# Autodesk Inventor assembly: Pulley
Saved by Autodesk Inventor 2016 (Build 200138000, 138)
## iProperties
Created: 2017-01-08
Part Number: Pulley
Document SubType Name: Assembly
Designer: Dhruv
Author: Dhruv
## Documents named in this file (4)
- C:\Users\Dhruv\Desktop\MISC\FRC 2017\Pulley.iam
- C:\Users\Dhruv\Desktop\MISC\FRC 2017\supporting_parts\am-2234_42toothHTDpulleyHalfRev2.ipt
- C:\Users\Dhruv\Desktop\MISC\FRC 2017\supporting_parts\am-2568 500EX Hex Hub.ipt
- C:\Users\Dhruv\Desktop\MISC\FRC 2017\HubBoltWithLockNut.iam
## Components (9 placed, 3 different names)
1. am-2234_42toothHTDpulleyHalfRev2:1
2. am-2234_42toothHTDpulleyHalfRev2:2
3. am-2568 500EX Hex Hub:1
4. HubBoltWithLockNut:1 [sub-assembly]
5. HubBoltWithLockNut:2 [sub-assembly]
6. HubBoltWithLockNut:3 [sub-assembly]
7. HubBoltWithLockNut:4 [sub-assembly]
8. HubBoltWithLockNut:5 [sub-assembly]
9. HubBoltWithLockNut:6 [sub-assembly]
## Relationships (19: Mate 19)
- [Mate]: am-2234_42toothHTDpulleyHalfRev2:1 ↔ am-2234_42toothHTDpulleyHalfRev2:2
- [Mate]: am-2234_42toothHTDpulleyHalfRev2:1 ↔ am-2234_42toothHTDpulleyHalfRev2:2
- [Mate]: am-2234_42toothHTDpulleyHalfRev2:1 ↔ am-2234_42toothHTDpulleyHalfRev2:2
- [Mate]: am-2234_42toothHTDpulleyHalfRev2:1 ↔ am-2234_42toothHTDpulleyHalfRev2:2
- [Mate]: am-2234_42toothHTDpulleyHalfRev2:2 ↔ am-2568 500EX Hex Hub:1
- [Mate]: am-2234_42toothHTDpulleyHalfRev2:2 ↔ am-2568 500EX Hex Hub:1
- [Mate]: am-2234_42toothHTDpulleyHalfRev2:2 ↔ am-2568 500EX Hex Hub:1
- [Mate]: am-2568 500EX Hex Hub:1 ↔ HubBoltWithLockNut:1
- [Mate]: am-2568 500EX Hex Hub:1 ↔ HubBoltWithLockNut:1
- [Mate]: am-2568 500EX Hex Hub:1 ↔ HubBoltWithLockNut:2
- [Mate]: am-2568 500EX Hex Hub:1 ↔ HubBoltWithLockNut:2
- [Mate]: am-2568 500EX Hex Hub:1 ↔ HubBoltWithLockNut:3
- [Mate]: am-2568 500EX Hex Hub:1 ↔ HubBoltWithLockNut:3
- [Mate]: am-2568 500EX Hex Hub:1 ↔ HubBoltWithLockNut:6
- [Mate]: am-2568 500EX Hex Hub:1 ↔ HubBoltWithLockNut:6
- [Mate]: am-2568 500EX Hex Hub:1 ↔ HubBoltWithLockNut:5
- [Mate]: am-2568 500EX Hex Hub:1 ↔ HubBoltWithLockNut:5
- [Mate]: am-2568 500EX Hex Hub:1 ↔ HubBoltWithLockNut:4
- [Mate]: am-2568 500EX Hex Hub:1 ↔ HubBoltWithLockNut:4
